# Autodesk Inventor assembly: ｍ2歯数13ギアd10甲ベアリング付き
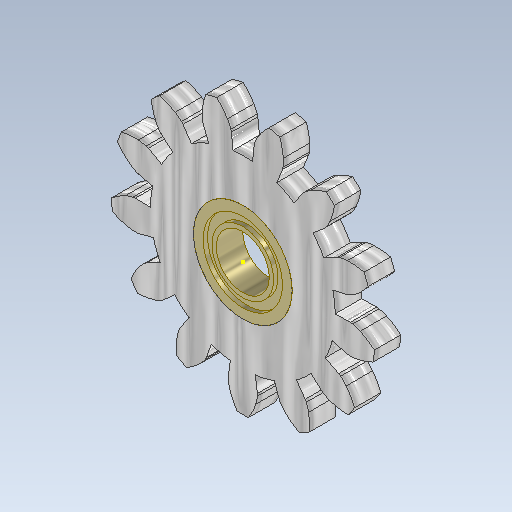
[picture p0: Inventor's stored thumbnail of the model, 512x512]
Saved by Autodesk Inventor 2020.2 (Build 242310000, 310)
## iProperties
Created: 2020-02-15
Part Number: ｍ2歯数13ギアd10甲ベアリング付き
Document SubType Name: Assembly
Designer: aoyam
Author: aoyam
## Documents named in this file (3)
- C:\Users\aoyam\Desktop\SRDC_local\Inventor\二年機\二年機インナー3層甲\ｍ2歯数13ギアd10甲ベアリング付き.iam
- C:\Users\aoyam\Desktop\SRDC_local\Inventor\二年機\二年機インナー3層甲\ｍ2歯数13ギアd10甲.ipt
- C:\Users\aoyam\Desktop\SRDC_local\Inventor\二年機\二年機インナー3層甲\ベアリングHd6-D10-B3甲.ipt
## Components (2 placed, 2 different names)
1. ｍ2歯数13ギアd10甲:1 — 挿入:1
2. ベアリングHd6-D10-B3甲:1 — 挿入:1
## Relationships (1: Insert 1)
- 挿入:1 [Insert]: ｍ2歯数13ギアd10甲:1 ↔ ベアリングHd6-D10-B3甲:1
